# Autodesk Inventor assembly: piMountForMeadeTripodLeg
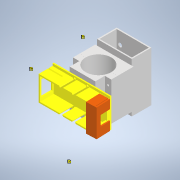
[picture p0: Inventor's stored thumbnail of the model, 180x180]
Saved by Autodesk Inventor 2021.2 (Build 252289000, 289)
## iProperties
Created: 2021-02-12
Part Number: piMountForMeadeTripodLeg
Document SubType Name: Assembly
Designer: robst
Author: robst
## Documents named in this file (6)
- C:\git\CAD-Development\robSteele\ShapeWays\TelescopeProjects\piMountForMeadeTripodLeg.iam
- C:\git\CAD-Development\robSteele\ShapeWays\TelescopeProjects\clampForMeadeTripodLeg.ipt
- C:\git\CAD-Development\robSteele\ShapeWays\TelescopeProjects\piCaseAttachesToTripodClamp.ipt
- C:\git\CAD-Development\robSteele\ShapeWays\TelescopeProjects\boltSideForclampForMeadeTripodLeg.ipt
- C:\git\CAD-Development\robSteele\ShapeWays\TelescopeProjects\usbHubCaseForTripodClamp.ipt
- C:\git\CAD-Development\robSteele\ShapeWays\TelescopeProjects\usbHubCaseTopChargingSide.ipt
## Components (5 placed, 5 different names)
1. clampForMeadeTripodLeg:1 — Insert:1, Insert:2, Insert:3, Insert:4
2. piCaseAttachesToTripodClamp:1 — Insert:1, Insert:2
3. boltSideForclampForMeadeTripodLeg:1 — Insert:3, Insert:4, Insert:5, Insert:6
4. usbHubCaseForTripodClamp:1 — Insert:5, Insert:6, Mate:1, Mate:2
5. usbHubCaseTopChargingSide:1 — Mate:1, Mate:2
## Relationships (8: Insert 6, Mate 2)
- Insert:1: clampForMeadeTripodLeg:1 ↔ piCaseAttachesToTripodClamp:1
- Insert:2: clampForMeadeTripodLeg:1 ↔ piCaseAttachesToTripodClamp:1
- Insert:3: clampForMeadeTripodLeg:1 ↔ boltSideForclampForMeadeTripodLeg:1
- Insert:4: clampForMeadeTripodLeg:1 ↔ boltSideForclampForMeadeTripodLeg:1
- Insert:5: boltSideForclampForMeadeTripodLeg:1 ↔ usbHubCaseForTripodClamp:1
- Insert:6: boltSideForclampForMeadeTripodLeg:1 ↔ usbHubCaseForTripodClamp:1
- Mate:1: usbHubCaseForTripodClamp:1 ↔ usbHubCaseTopChargingSide:1
- Mate:2: usbHubCaseForTripodClamp:1 ↔ usbHubCaseTopChargingSide:1
